# Autodesk Inventor assembly: Limit switch bottom + mount right
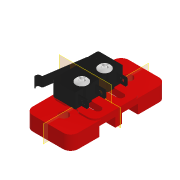
[picture p0: Inventor's stored thumbnail of the model, 180x180]
Saved by Autodesk Inventor 2020 (Build 240168000, 168)
## iProperties
Created: 2020-01-01
Part Number: Limit switch bottom + mount right
Document SubType Name: Assembly
Designer: ball
Author: ball
## Documents named in this file (5)
- C:\FTC\FTC8863CAD\2019 Robot\Delivery\Lift Right\Limit switch bottom + mount right.iam
- C:\FTC\FTC8863CAD\2019 Robot\Generic Parts\limit switch mount to xrail.ipt
- C:\FTC\FTC8863CAD\Actobotics\605 parts\605632.ipt
- C:\FTC\FTC8863CAD\StepLibraries\Nuts\2-56 NYLON-INSERT LOCKNUT.ipt
- C:\FTC\FTC8863CAD\StepLibraries\Screws\2-56 x .5 TRUSS HEAD PHILLIPS MACHINE SCREW.ipt
## Components (6 placed, 4 different names)
1. limit switch mount to xrail:1 — Mate:1, Flush:1, Flush:2, Mate:2, Angle:1, Mate:4, Angle:2
2. 605632:1 — Mate:1, Flush:1, Flush:2, Mate:3, Mate:5, Mate:6, Mate:7, Mate:8, Mate:9
3. 2-56 NYLON-INSERT LOCKNUT:1 — Mate:2, Mate:3, Angle:1
4. 2-56 NYLON-INSERT LOCKNUT:2 — Mate:4, Mate:5, Angle:2
5. 2-56 x .5 TRUSS HEAD PHILLIPS MACHINE SCREW:1 — Mate:6, Mate:7
6. 2-56 x .5 TRUSS HEAD PHILLIPS MACHINE SCREW:2 — Mate:8, Mate:9
## Relationships (13: Mate 9, Flush 2, Angle 2)
- Mate:1: limit switch mount to xrail:1 ↔ 605632:1
- Flush:1 (1.27 mm): limit switch mount to xrail:1 ↔ 605632:1
- Flush:2: limit switch mount to xrail:1 ↔ 605632:1
- Mate:2: limit switch mount to xrail:1 ↔ 2-56 NYLON-INSERT LOCKNUT:1
- Mate:3: 605632:1 ↔ 2-56 NYLON-INSERT LOCKNUT:1
- Angle:1 (0 deg): limit switch mount to xrail:1 ↔ 2-56 NYLON-INSERT LOCKNUT:1
- Mate:4: limit switch mount to xrail:1 ↔ 2-56 NYLON-INSERT LOCKNUT:2
- Mate:5: 605632:1 ↔ 2-56 NYLON-INSERT LOCKNUT:2
- Angle:2 (0 deg): limit switch mount to xrail:1 ↔ 2-56 NYLON-INSERT LOCKNUT:2
- Mate:6: 605632:1 ↔ 2-56 x .5 TRUSS HEAD PHILLIPS MACHINE SCREW:1
- Mate:7: 605632:1 ↔ 2-56 x .5 TRUSS HEAD PHILLIPS MACHINE SCREW:1
- Mate:8: 605632:1 ↔ 2-56 x .5 TRUSS HEAD PHILLIPS MACHINE SCREW:2
- Mate:9: 605632:1 ↔ 2-56 x .5 TRUSS HEAD PHILLIPS MACHINE SCREW:2
